# Autodesk Inventor assembly: MGN07C_1_R_80_ZF_H_M_1
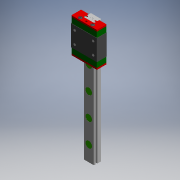
[picture p0: Inventor's stored thumbnail of the model, 180x180]
Saved by Autodesk Inventor 2016 (Build 200138000, 138)
## iProperties
Company: CADClick - KiM GmbH - www.kimweb.de
Created: 2015-04-23
Part Number: MGN07C_1_R_80_ZF_H_M_1
Description: no description
Document SubType Name: Assembly
Designer: ax
Authority: unknown authorization
Sending System: ACIS
Preprocessor: unknown preprocess
Title: MGN07C_1_R_80_ZF_H_M_1.stp
Author: HIWIN GmbH
## Documents named in this file (3)
- C:\Users\ax\Documents\Inventor\mintplacer\MGN07C_1_R_80_ZF_H_M_1.iam
- C:\Users\ax\Documents\Inventor\mintplacer\1.ipt
- C:\Users\ax\Documents\Inventor\mintplacer\2.ipt
## Components (2 placed, 2 different names)
1. MGN7C carriage — Slider:1
2. MGN7 rail — Slider:1
## Relationships (1: TranslationJoint 1)
- Slider:1 [TranslationJoint]: MGN7C carriage ↔ MGN7 rail
